# Autodesk Inventor assembly: Mic_Array_Complete
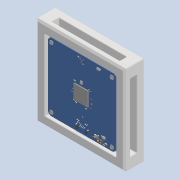
[picture p0: Inventor's stored thumbnail of the model, 180x180]
Saved by Autodesk Inventor 2020 (Build 240168000, 168)
## iProperties
Created: 2020-08-27
Part Number: Mic_Array_Complete
Document SubType Name: Assembly
Designer: conno
Author: conno
## Documents named in this file (5)
- C:\Users\conno\Documents\Clients\flatearth\NIH\GitHub\hardware\Projects\AB_Mic_Array\Housing\Mic_Array_Complete.iam
- C:\Users\conno\Documents\Clients\flatearth\NIH\GitHub\hardware\Projects\AB_Mic_Array\Housing\PCB\Audio Blade Microphone Array 0P1.iam
- C:\Users\conno\Documents\Clients\flatearth\NIH\GitHub\hardware\Projects\AB_Mic_Array\Housing\Components\92095A177_BUTTON HEAD HEX DRIVE SCREW.ipt
- C:\Users\conno\Documents\Clients\flatearth\NIH\GitHub\hardware\Projects\AB_Mic_Array\Housing\Bracket\Back_Plate.ipt
- C:\Users\conno\Documents\Clients\flatearth\NIH\GitHub\hardware\Projects\AB_Mic_Array\Housing\Bracket\Face_Plate.ipt
## Components (7 placed, 4 different names)
1. Audio Blade Microphone Array 0P1:1 [sub-assembly] — Mate:4, Mate:6, Mate:7, Mate:8, Mate:9, Mate:10, Mate:11
2. 92095A177_BUTTON HEAD HEX DRIVE SCREW:1 — Mate:4
3. 92095A177_BUTTON HEAD HEX DRIVE SCREW:2 — Mate:6, Mate:7
4. 92095A177_BUTTON HEAD HEX DRIVE SCREW:3 — Mate:8, Mate:9
5. 92095A177_BUTTON HEAD HEX DRIVE SCREW:4 — Mate:10, Mate:11
6. Back_Plate:1 — Mate:12, Flush:1, Mate:13
7. Face_Plate:1 — Mate:12, Flush:1, Mate:13
## Relationships (10: Mate 9, Flush 1)
- Mate:4: Audio Blade Microphone Array 0P1:1 ↔ 92095A177_BUTTON HEAD HEX DRIVE SCREW:1
- Mate:6: Audio Blade Microphone Array 0P1:1 ↔ 92095A177_BUTTON HEAD HEX DRIVE SCREW:2
- Mate:7: Audio Blade Microphone Array 0P1:1 ↔ 92095A177_BUTTON HEAD HEX DRIVE SCREW:2
- Mate:8: Audio Blade Microphone Array 0P1:1 ↔ 92095A177_BUTTON HEAD HEX DRIVE SCREW:3
- Mate:9: Audio Blade Microphone Array 0P1:1 ↔ 92095A177_BUTTON HEAD HEX DRIVE SCREW:3
- Mate:10: Audio Blade Microphone Array 0P1:1 ↔ 92095A177_BUTTON HEAD HEX DRIVE SCREW:4
- Mate:11: Audio Blade Microphone Array 0P1:1 ↔ 92095A177_BUTTON HEAD HEX DRIVE SCREW:4
- Mate:12: Back_Plate:1 ↔ Face_Plate:1
- Flush:1: Back_Plate:1 ↔ Face_Plate:1
- Mate:13: Back_Plate:1 ↔ Face_Plate:1
